# Autodesk Inventor assembly: ASY NVPH-466 joint flange
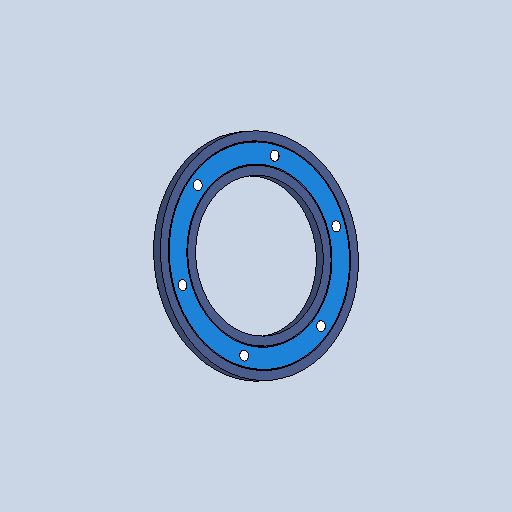
[picture p0: Inventor's stored thumbnail of the model, 512x512]
Saved by Autodesk Inventor 2025.1 (Build 291241020, 241B)
## iProperties
Created: 2024-12-03
Part Number: ASY NVPH-466 joint flange
Document SubType Name: Assembly
Designer: admin
Author: admin
## Documents named in this file (4)
- C:\Users\user\YandexDisk-badmisterfox\домашниий пк\Inventor\NDM-VOS_powder_hopper\ASY NVPH-466 joint flange.iam
- C:\Users\user\YandexDisk-badmisterfox\домашниий пк\Inventor\NDM-VOS_powder_hopper\NVPH-413 revision steel circle.ipt
- C:\Users\user\YandexDisk-badmisterfox\домашниий пк\Inventor\NDM-VOS_powder_hopper\NVPH-412 revision plastic circle.ipt
- C:\Users\user\YandexDisk-badmisterfox\домашниий пк\Inventor\Content Center Files\en-US\DIN 976-1 A\DIN 976-1 - M10 x 30 - A.ipt
## Components (8 placed, 3 different names)
1. NVPH-413 revision steel circle.ipt:1
2. NVPH-412 revision plastic circle.ipt:1
3. DIN 976-1 - M10 x 30 - A.ipt:1
4. DIN 976-1 - M10 x 30 - A.ipt:2
5. DIN 976-1 - M10 x 30 - A.ipt:3
6. DIN 976-1 - M10 x 30 - A.ipt:4
7. DIN 976-1 - M10 x 30 - A.ipt:5
8. DIN 976-1 - M10 x 30 - A.ipt:6
## Relationships (6: RevoluteJoint 6)
- [RevoluteJoint]: NVPH-413 revision steel circle.ipt:1 ↔ DIN 976-1 - M10 x 30 - A.ipt:1
- [RevoluteJoint]: NVPH-413 revision steel circle.ipt:1 ↔ DIN 976-1 - M10 x 30 - A.ipt:2
- [RevoluteJoint]: NVPH-413 revision steel circle.ipt:1 ↔ DIN 976-1 - M10 x 30 - A.ipt:3
- [RevoluteJoint]: NVPH-413 revision steel circle.ipt:1 ↔ DIN 976-1 - M10 x 30 - A.ipt:6
- [RevoluteJoint]: NVPH-413 revision steel circle.ipt:1 ↔ DIN 976-1 - M10 x 30 - A.ipt:4
- [RevoluteJoint]: NVPH-413 revision steel circle.ipt:1 ↔ DIN 976-1 - M10 x 30 - A.ipt:5
